# Autodesk Inventor assembly: Body
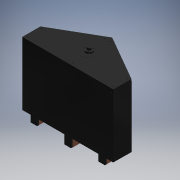
[picture p0: Inventor's stored thumbnail of the model, 180x180]
Saved by Autodesk Inventor 2017 (Build 210142000, 142)
## iProperties
Created: 2018-10-18
Part Number: Body
Document SubType Name: Assembly
Designer: Dell
Author: Dell
## Documents named in this file (6)
- C:\Users\Dell\Documents\GitHub\tr2\Body\Body.iam
- C:\Users\Dell\Documents\GitHub\tr2\Body\Body Cover Assembly.iam
- C:\Users\Dell\Documents\GitHub\tr2\Body\Body Chassis Assembly.iam
- C:\Users\Dell\Documents\GitHub\tr2\Base\37d-gearmotor-50-70-encoder.ipt
- C:\Users\Dell\Documents\GitHub\tr2\Arm Actuator\Arm Actuator.iam
- C:\Users\Dell\Documents\GitHub\tr2\Body\BO13.ipt
## Components (5 placed, 5 different names)
1. Body Cover Assembly:1 [sub-assembly] — Mate:63, Mate:64, Mate:65
2. Body Chassis Assembly:1 [sub-assembly] — Mate:59, Mate:60, Mate:61, Mate:62, Mate:63, Mate:64, Mate:65, Flush:2, Mate:67, Mate:68
3. 37d-gearmotor-50-70-encoder:1 — Mate:66
4. Arm Actuator:1 [sub-assembly] — Flush:2, Mate:66, Mate:69, Mate:70, Mate:71
5. BO13:1 — Mate:67, Mate:68, Mate:69, Mate:70, Mate:71
## Relationships (14: Mate 13, Flush 1)
- Mate:59: Body Chassis Assembly:1
- Mate:60: Body Chassis Assembly:1
- Mate:61: Body Chassis Assembly:1
- Mate:62: Body Chassis Assembly:1
- Mate:63: Body Cover Assembly:1 ↔ Body Chassis Assembly:1
- Mate:64: Body Cover Assembly:1 ↔ Body Chassis Assembly:1
- Mate:65: Body Cover Assembly:1 ↔ Body Chassis Assembly:1
- Flush:2 (-10 mm): Body Chassis Assembly:1 ↔ Arm Actuator:1
- Mate:66: 37d-gearmotor-50-70-encoder:1 ↔ Arm Actuator:1
- Mate:67: Body Chassis Assembly:1 ↔ BO13:1
- Mate:68: Body Chassis Assembly:1 ↔ BO13:1
- Mate:69: Arm Actuator:1 ↔ BO13:1
- Mate:70: Arm Actuator:1 ↔ BO13:1
- Mate:71: Arm Actuator:1 ↔ BO13:1
